# Autodesk Inventor assembly: Zonnepaneel V5.0
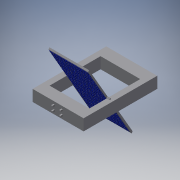
[picture p0: Inventor's stored thumbnail of the model, 180x180]
Saved by Autodesk Inventor 2018.3 (Build 223284000, 284)
## iProperties
Created: 2020-11-27
Part Number: Zonnepaneel V5.0
Document SubType Name: Assembly
Designer: daanv
Author: daanv
## Documents named in this file (3)
- C:\Users\daanv\OneDrive\Documenten\Life\Avans Project RED\Gebouw\Zonnepaneel V5.0.iam
- C:\Users\daanv\OneDrive\Documenten\Life\Avans Project RED\Gebouw\Frame V2.ipt
- C:\Users\daanv\OneDrive\Documenten\Life\Avans Project RED\Gebouw\Zonnepaneel V5.0.ipt
## Components (2 placed, 2 different names)
1. Frame V2:1 — Mate:3, Mate:4
2. Zonnepaneel V5.0:1 — Mate:3, Mate:4
## Relationships (2: Mate 2)
- Mate:3: Frame V2:1 ↔ Zonnepaneel V5.0:1
- Mate:4: Frame V2:1 ↔ Zonnepaneel V5.0:1
